# Autodesk Inventor assembly: 4K shield2
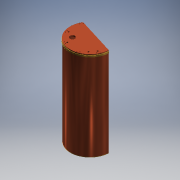
[picture p0: Inventor's stored thumbnail of the model, 180x180]
Saved by Autodesk Inventor 2018 (Build 220112000, 112)
## iProperties
Created: 2019-03-11
Part Number: 4K shield2
Document SubType Name: Assembly
Designer: Admin
Author: Admin
## Documents named in this file (7)
- C:\Users\Admin\Documents\Cryostat\CAD\4K shield2.iam
- C:\Users\Admin\Documents\Cryostat\CAD\4K sheild body2.ipt
- C:\Users\Admin\Documents\Cryostat\CAD\4K sheild rim3.ipt
- C:\Users\Admin\Documents\Cryostat\CAD\4K shield bottom.ipt
- C:\Users\Admin\Documents\Cryostat\CAD\4K shield cover.ipt
- C:\Users\Admin\Documents\Cryostat\CAD\4K adapter.ipt
- C:\Users\Admin\Documents\Cryostat\CAD\4K sheild top.ipt
## Components (13 placed, 6 different names)
1. 4K shield bottom:1 — Mate:6, Mate:7, Mate:8, Mate:39, Mate:40
2. 4K shield cover:1 — Mate:6, Mate:7, Mate:8
3. 4K adapter:1 — Flush:3, Flush:7, Mate:21, Mate:22
4. 4K adapter:2 — Flush:4, Mate:17, Mate:18
5. 4K adapter:3 — Flush:7, Mate:19, Mate:20
6. 4K adapter:4 — Flush:1, Flush:4, Mate:31, Mate:32, Mate:33, Mate:35
7. 4K adapter:5 — Flush:5, Mate:25, Mate:29
8. 4K adapter:6 — Flush:6, Mate:23, Mate:27, Mate:34
9. 4K adapter:7 — Flush:2, Flush:3, Flush:6, Mate:24, Mate:28
10. 4K adapter:8 — Flush:1, Flush:2, Flush:5, Mate:26, Mate:30
11. 4K sheild top:1 — Mate:17, Mate:18, Mate:19, Mate:20, Mate:21, Mate:22, Mate:23, Mate:24, Mate:25, Mate:26, Mate:27, Mate:28, Mate:29, Mate:30, Mate:31, Mate:32, Mate:33, Mate:36
12. 4K sheild rim3:1 — Mate:34, Mate:35, Mate:36, Mate:37, Mate:38
13. 4K sheild body2:1 — Mate:37, Mate:38, Mate:39, Mate:40
## Relationships (34: Mate 27, Flush 7)
- Mate:6: 4K shield bottom:1 ↔ 4K shield cover:1
- Mate:7: 4K shield bottom:1 ↔ 4K shield cover:1
- Mate:8: 4K shield bottom:1 ↔ 4K shield cover:1
- Flush:1: 4K adapter:4 ↔ 4K adapter:8
- Flush:2: 4K adapter:7 ↔ 4K adapter:8
- Flush:3: 4K adapter:1 ↔ 4K adapter:7
- Flush:4: 4K adapter:2 ↔ 4K adapter:4
- Flush:5: 4K adapter:5 ↔ 4K adapter:8
- Flush:6: 4K adapter:6 ↔ 4K adapter:7
- Flush:7: 4K adapter:1 ↔ 4K adapter:3
- Mate:17: 4K adapter:2 ↔ 4K sheild top:1
- Mate:18: 4K adapter:2 ↔ 4K sheild top:1
- Mate:19: 4K adapter:3 ↔ 4K sheild top:1
- Mate:20: 4K adapter:3 ↔ 4K sheild top:1
- Mate:21: 4K adapter:1 ↔ 4K sheild top:1
- Mate:22: 4K adapter:1 ↔ 4K sheild top:1
- Mate:23: 4K adapter:6 ↔ 4K sheild top:1
- Mate:24: 4K adapter:7 ↔ 4K sheild top:1
- Mate:25: 4K adapter:5 ↔ 4K sheild top:1
- Mate:26: 4K adapter:8 ↔ 4K sheild top:1
- Mate:27: 4K adapter:6 ↔ 4K sheild top:1
- Mate:28: 4K adapter:7 ↔ 4K sheild top:1
- Mate:29: 4K adapter:5 ↔ 4K sheild top:1
- Mate:30: 4K adapter:8 ↔ 4K sheild top:1
- Mate:31: 4K adapter:4 ↔ 4K sheild top:1
- Mate:32: 4K adapter:4 ↔ 4K sheild top:1
- Mate:33: 4K adapter:4 ↔ 4K sheild top:1
- Mate:34: 4K adapter:6 ↔ 4K sheild rim3:1
- Mate:35: 4K adapter:4 ↔ 4K sheild rim3:1
- Mate:36: 4K sheild top:1 ↔ 4K sheild rim3:1
- Mate:37: 4K sheild rim3:1 ↔ 4K sheild body2:1
- Mate:38: 4K sheild rim3:1 ↔ 4K sheild body2:1
- Mate:39: 4K shield bottom:1 ↔ 4K sheild body2:1
- Mate:40: 4K shield bottom:1 ↔ 4K sheild body2:1
